# Autodesk Inventor assembly: CA23[F]
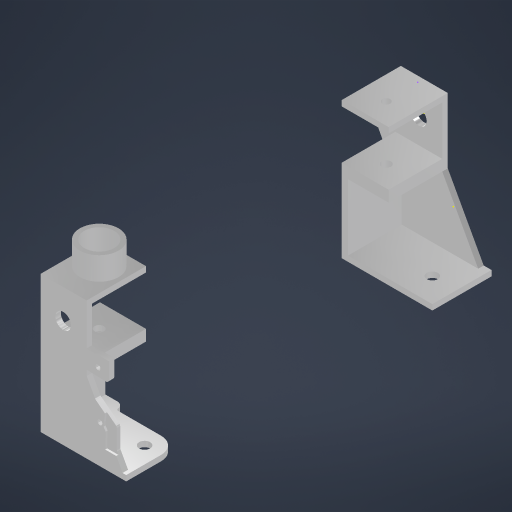
[picture p0: Inventor's stored thumbnail of the model, 512x512]
Saved by Autodesk Inventor 2023 (Build 270158000, 158)
## iProperties
Created: 2023-01-25
Part Number: CA23[F]
Document SubType Name: Assembly
Designer: juanj
Author: juanj
## Documents named in this file (5)
- C:\Users\juanj\OneDrive\Documentos\Unisabana\Shell\C23 DESING\A23[i2]\CA23[F].iam
- C:\Users\juanj\OneDrive\Documentos\Unisabana\Shell\C23 DESING\A23[i2]\AC23[i3][L].ipt
- C:\Users\juanj\OneDrive\Documentos\Unisabana\Shell\C23 DESING\A23[i2]\AC23[I3][R].ipt
- C:\Users\juanj\OneDrive\Documentos\Unisabana\Shell\C23 DESING\A23[i2]\C23[i3][L].ipt
- C:\Users\juanj\OneDrive\Documentos\Unisabana\Shell\C23 DESING\A23[i2]\C23[i3][R].ipt
## Components (4 placed, 4 different names)
1. AC23[i3][L]:1 — Insertar:1, Ángulo:1, Nivelación:1, Nivelación:2
2. AC23[I3][R]:1 — Insertar:2, Ángulo:2, Nivelación:1, Nivelación:2
3. C23[i3][L]:1 — Insertar:1, Ángulo:1, Ángulo:3
4. C23[i3][R]:1 — Insertar:2, Ángulo:2, Ángulo:3
## Relationships (7: Angle 3, Insert 2, Flush 2)
- Insertar:1: AC23[i3][L]:1 ↔ C23[i3][L]:1
- Ángulo:1 [Angle] (0 deg): AC23[i3][L]:1 ↔ C23[i3][L]:1
- Insertar:2: AC23[I3][R]:1 ↔ C23[i3][R]:1
- Ángulo:2 [Angle] (0 deg): AC23[I3][R]:1 ↔ C23[i3][R]:1
- Ángulo:3 [Angle] (0 deg): C23[i3][L]:1 ↔ C23[i3][R]:1
- Nivelación:1 [Flush]: AC23[i3][L]:1 ↔ AC23[I3][R]:1
- Nivelación:2 [Flush]: AC23[i3][L]:1 ↔ AC23[I3][R]:1
